# Autodesk Inventor assembly: Hand-w-Specialty_Gussets
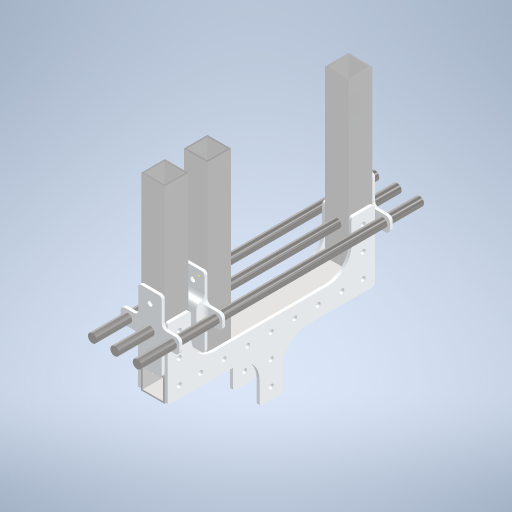
[picture p0: Inventor's stored thumbnail of the model, 512x512]
Saved by Autodesk Inventor 2024 (Build 280153000, 153)
## iProperties
Created: 2024-01-20
Part Number: Hand-w-Specialty_Gussets
Document SubType Name: Assembly
Designer: aidan
Author: aidan
## Documents named in this file (7)
- C:\Users\aidan\OneDrive\Documents\Inventor\Content Center Files\Hand-w-Specialty_Gussets.iam
- C:\Users\aidan\OneDrive\Documents\Inventor\Content Center Files\Tube Finger.ipt
- C:\Users\aidan\OneDrive\Documents\Inventor\Content Center Files\Lead Nut Holder Mk2.ipt
- C:\Users\aidan\OneDrive\Documents\Inventor\Content Center Files\Guide Rod Holder.ipt
- C:\Users\aidan\OneDrive\Documents\Inventor\Content Center Files\Finger Base.ipt
- C:\Users\aidan\OneDrive\Documents\Inventor\Content Center Files\Lead_Shaft.ipt
- C:\Users\aidan\OneDrive\Documents\Inventor\Content Center Files\Specialty Arm Gusset.ipt
## Components (12 placed, 6 different names)
1. Tube Finger:1 — Mate:1, Rotational:3
2. Tube Finger:2 — Mate:1
3. Lead Nut Holder Mk2:1
4. Tube Finger:3 — Rotational:7
5. Guide Rod Holder:1 — Rotational:3
6. Finger Base:1 — Rotational:11, Rotational:12
7. Guide Rod Holder:2 — Rotational:7, Rotational:8, Rotational:9, Rotational:10
8. Lead_Shaft:1 — Rotational:10
9. Lead_Shaft:2 — Rotational:9
10. Lead_Shaft:3 — Rotational:8
11. Specialty Arm Gusset:1 — Rotational:12
12. Specialty Arm Gusset:2 — Rotational:11
## Relationships (8: RevoluteJoint 7, Mate 1)
- Mate:1 (127 mm): Tube Finger:1 ↔ Tube Finger:2
- Rotational:3 [RevoluteJoint]: Tube Finger:1 ↔ Guide Rod Holder:1
- Rotational:7 [RevoluteJoint]: Tube Finger:3 ↔ Guide Rod Holder:2
- Rotational:8 [RevoluteJoint] (-38.1 mm): Guide Rod Holder:2 ↔ Lead_Shaft:3
- Rotational:9 [RevoluteJoint] (-38.1 mm): Guide Rod Holder:2 ↔ Lead_Shaft:2
- Rotational:10 [RevoluteJoint] (-38.1 mm): Guide Rod Holder:2 ↔ Lead_Shaft:1
- Rotational:11 [RevoluteJoint]: Finger Base:1 ↔ Specialty Arm Gusset:2
- Rotational:12 [RevoluteJoint]: Finger Base:1 ↔ Specialty Arm Gusset:1
